# Autodesk Inventor assembly: AM14U2 Half Long
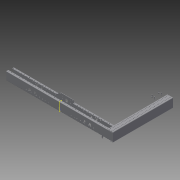
[picture p0: Inventor's stored thumbnail of the model, 180x180]
Saved by Autodesk Inventor 2015 (Build 190159000, 159)
## iProperties
Created: 2015-01-10
Part Number: AM14U2 Half Long
Document SubType Name: Assembly
Designer: whitaus15
Author: whitaus15
## Documents named in this file (5)
- \\lhssvr02\Homedirs\Robotics Club\CAD Model 2015\Imported Components\AM14U2 Long\AM14U2 Half Long.iam
- \\lhssvr02\Homedirs\Robotics Club\CAD Model 2015\Imported Components\AM14U2 Long\am-2951 AM14U2 Outside Sheet.ipt
- \\lhssvr02\Homedirs\Robotics Club\CAD Model 2015\Imported Components\AM14U2 Long\Sheet Metal Front-Back.ipt
- \\lhssvr02\Homedirs\Robotics Club\CAD Model 2015\Imported Components\AM14U2 Long\10-32x0625 with nut.iam
- \\lhssvr02\Homedirs\Robotics Club\CAD Model 2015\Imported Components\AM14U2 Long\am-2952 AM14U2 Inside Sheet Mod.ipt
## Components (15 placed, 15 different names)
1. am-2951 AM14U2 Outside Sheet_9 — Flush:1, Flush:2, Mate:1
2. am-2952 AM14U2 Inside Sheet_10 — Tangent:1, Mate:2
3. Sheet Metal Front-Back_19 — Flush:1, Flush:2, Mate:1, Tangent:1, Mate:2
4. 10-32x0625 with nut_22 [sub-assembly]
5. 10-32x0625 with nut_23 [sub-assembly]
6. 10-32x0625 with nut_24 [sub-assembly]
7. 10-32x0625 with nut_25 [sub-assembly]
8. 10-32x0625 with nut_26 [sub-assembly]
9. 10-32x0625 with nut_27 [sub-assembly]
10. 10-32x0625 with nut_28 [sub-assembly]
11. 10-32x0625 with nut_29 [sub-assembly]
12. 10-32x0625 with nut_30 [sub-assembly]
13. 10-32x0625 with nut_31 [sub-assembly]
14. 10-32x0625 with nut_32 [sub-assembly]
15. 10-32x0625 with nut_33 [sub-assembly]
## Relationships (5: Flush 2, Mate 2, Tangent 1)
- Flush:1: am-2951 AM14U2 Outside Sheet_9 ↔ Sheet Metal Front-Back_19
- Flush:2: am-2951 AM14U2 Outside Sheet_9 ↔ Sheet Metal Front-Back_19
- Mate:1: am-2951 AM14U2 Outside Sheet_9 ↔ Sheet Metal Front-Back_19
- Tangent:1: am-2952 AM14U2 Inside Sheet_10 ↔ Sheet Metal Front-Back_19
- Mate:2: am-2952 AM14U2 Inside Sheet_10 ↔ Sheet Metal Front-Back_19
